# Autodesk Inventor assembly: standoff_bracce
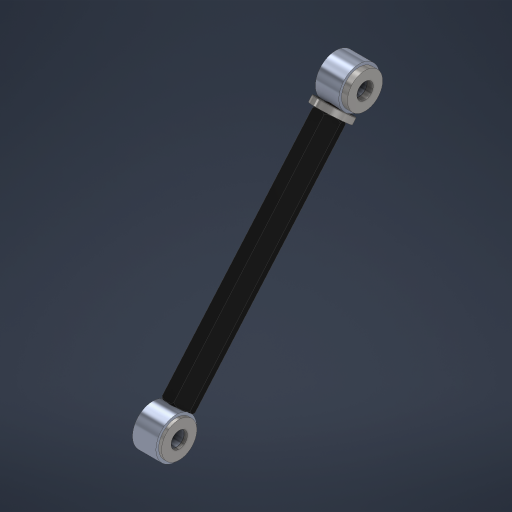
[picture p0: Inventor's stored thumbnail of the model, 512x512]
Saved by Autodesk Inventor 2024 (Build 280153000, 153)
## iProperties
Created: 2023-10-19
Part Number: standoff_bracce
Document SubType Name: Assembly
Designer: Averey Ku
Author: Averey Ku
## Documents named in this file (7)
- D:\vex_robotics\hardware\cad\goated_v0.1\catapult\standoff_bracce.iam
- D:\vex_robotics\hardware\cad\VEX-CAD-Inventor-1.41\Structure\Standoff\Standoff 2.50.ipt
- D:\vex_robotics\hardware\cad\VEX-CAD-Inventor-1.41\Structure\Standoff.ipt
- D:\vex_robotics\hardware\cad\VEX-CAD-Inventor-1.41\Motion\Shaft LS\Shaft Collar ipts\Shaft Collar No Screw.ipt
- D:\vex_robotics\hardware\cad\VEX-CAD-Inventor-1.41\Motion\Spacers\Washer Steel\SWasher .375 OD x .062500.ipt
- D:\vex_robotics\hardware\cad\VEX-CAD-Inventor-1.41\Motion\Spacers\Washer Steel.ipt
- D:\vex_robotics\hardware\cad\VEX-CAD-Inventor-1.41\Motion\Spacers\Washer Steel\SWasher .375 OD x .031250.ipt
## Components (6 placed, 4 different names)
1. Standoff 2.50:1 — Mate:1, Insert:3
2. Shaft Collar No Screw:1 — Mate:1, Insert:2
3. Shaft Collar No Screw:2 — Insert:1, Insert:4
4. SWasher .375 OD x .062500:1 — Insert:3, Insert:4
5. SWasher .375 OD x .062500:2 — Insert:1
6. SWasher .375 OD x .031250:3 — Insert:2
## Relationships (5: Insert 4, Mate 1)
- Mate:1: Standoff 2.50:1 ↔ Shaft Collar No Screw:1
- Insert:1: Shaft Collar No Screw:2 ↔ SWasher .375 OD x .062500:2
- Insert:2: Shaft Collar No Screw:1 ↔ SWasher .375 OD x .031250:3
- Insert:3: Standoff 2.50:1 ↔ SWasher .375 OD x .062500:1
- Insert:4: Shaft Collar No Screw:2 ↔ SWasher .375 OD x .062500:1
